# Autodesk Inventor assembly: Plate
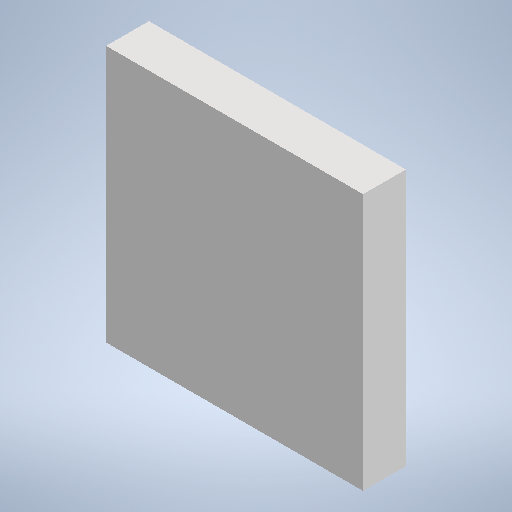
[picture p0: Inventor's stored thumbnail of the model, 512x512]
Saved by Autodesk Inventor 2026 (Build 300175050, 175E)
## iProperties
Created: 2026-01-31
Part Number: Plate
Document SubType Name: Assembly
Designer: TiffanyHayden
Author: TiffanyHayden
## Documents named in this file (2)
- C:\Users\TiffanyHayden\Documents\GitHub\CodingCADventure\CodingCADventureCSharp\CodingCADventureCSharp\InventorFiles\Plate.iam
- C:\Users\TiffanyHayden\Documents\GitHub\CodingCADventure\CodingCADventureCSharp\CodingCADventureCSharp\InventorFiles\Plate.ipt
## Components (1 placed, 1 different names)
1. Plate:1 — Flush:2, Flush:3, Flush:4
## Relationships (3: Flush 3)
- Flush:2: Plate:1
- Flush:3: Plate:1
- Flush:4: Plate:1
